# Autodesk Inventor assembly: panTiltSystemRB02
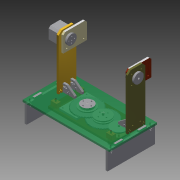
[picture p0: Inventor's stored thumbnail of the model, 180x180]
Saved by Autodesk Inventor 2013 (Build 170138000, 138)
## iProperties
Created: 2014-06-24
Part Number: panTiltSystemRB02
Document SubType Name: Assembly
Designer: Nano
Author: Nano
## Documents named in this file (23)
- C:\Users\Nano\Documents\InventorByron\InventorMasterProject\panTiltSystem\panTiltSystemRB02.iam
- C:\Users\Nano\Documents\InventorByron\InventorMasterProject\panTiltSystem\baseBoxShortSideRB01.ipt
- C:\Users\Nano\Documents\InventorByron\InventorMasterProject\panTiltSystem\panStepperMountRB01.ipt
- C:\Users\Nano\Documents\InventorByron\InventorMasterProject\panTiltSystem\stepper42BYGH007_RB01.ipt
- C:\Users\Nano\Documents\InventorByron\InventorMasterProject\panTiltSystem\tiltStructureCrossBeamRB01.ipt
- C:\Users\Nano\Documents\InventorByron\InventorMasterProject\panTiltSystem\tiltColumnStepperSide02_RB01.ipt
- C:\Users\Nano\Documents\InventorByron\InventorMasterProject\panTiltSystem\tiltColumnNonStepperSide02_RB01.ipt
- C:\Users\Nano\Documents\InventorByron\InventorMasterProject\panTiltSystem\projectorMountSide_RB01.ipt
- C:\Users\Nano\Documents\InventorByron\InventorMasterProject\panTiltSystem\projectorMountingBase_RB01.ipt
- C:\Users\Nano\Documents\InventorByron\InventorMasterProject\panTiltSystem\stepperShaftCollar_RB01.ipt
- C:\Users\Nano\Documents\InventorByron\InventorMasterProject\panTiltSystem\projectorMountOppositeSide_RB01.ipt
- C:\Users\Nano\Documents\InventorByron\InventorMasterProject\panTiltSystem\rotatingSupportShaft_RB01.ipt
- C:\Users\Nano\Documents\InventorByron\InventorMasterProject\panTiltSystem\shaftEndPlate_RB01.ipt
- C:\Users\Nano\Documents\InventorByron\InventorMasterProject\panTiltSystem\aaxaProjector01_RB01.ipt
- C:\Users\Nano\Documents\InventorByron\InventorMasterProject\panTiltSystem\cornerBraceV01.ipt
- C:\Users\Nano\Documents\InventorByron\InventorMasterProject\panTiltSystem\gearExperiments\gearTry01.iam
- C:\Users\Nano\Documents\InventorByron\InventorMasterProject\panTiltSystem\panGearShaft1.ipt
- C:\Users\Nano\Documents\InventorByron\InventorMasterProject\panTiltSystem\panGearSpacerBlocks.ipt
- C:\Users\Nano\Documents\InventorByron\InventorMasterProject\panTiltSystem\gearSpacerDisc01.ipt
- C:\Users\Nano\Documents\InventorByron\InventorMasterProject\panTiltSystem\gearGuideDiscOutputStage1.ipt
- C:\Users\Nano\Documents\InventorByron\InventorMasterProject\panTiltSystem\gearSpacerSmallOutputStage.ipt
- C:\Users\Nano\Documents\InventorByron\InventorMasterProject\panTiltSystem\panTilt_RB02_cutFiles\cutFiles125\driveGearCap.ipt
- C:\Users\Nano\Documents\InventorByron\InventorMasterProject\panTiltSystem\panTilt_RB02_cutFiles\cutFiles125\outputGearSupport.ipt
## Components (35 placed, 22 different names)
1. baseBoxShortSideRB01:1 — Mate:2, Flush:3, Mate:4
2. baseBoxShortSideRB01:2 — Mate:1, Mate:1, Flush:2
3. panStepperMountRB01:1 — Mate:1, Mate:1, Flush:2, Mate:2, Flush:3, Mate:4, Mate:7, Mate:60, Mate:61, Angle:6, Mate:64, Mate:72, Flush:27, Flush:28
4. stepper42BYGH007_RB01:1 — Mate:9, Mate:10, Mate:12, Mate:25, Mate:28, Mate:29, Mate:31, Mate:33
5. stepper42BYGH007_RB01:2 — zeroPositionPan, zeroPositionTilt, Mate:62, Mate:63
6. tiltStructureCrossBeamRB01:1 — Mate:7, Flush:5, Mate:8, Flush:6, Mate:11, Flush:7, Mate:15, Mate:18, Mate:21, Mate:24, Mate:48, Mate:50, Mate:51, Mate:54, Mate:56
7. tiltColumnStepperSide02_RB01:1 — Flush:5, Mate:8, Flush:6, Mate:9, Mate:10, Mate:28, Mate:32, Mate:49, Mate:52, Mate:53
8. tiltColumnNonStepperSide02_RB01:1 — Mate:11, Mate:12, Flush:7, Mate:39, zeroPositionPan, Mate:55, Mate:57, Mate:58, Mate:59
9. cornerBraceV01:1 — Mate:48, Mate:49, Flush:17
10. cornerBraceV01:2 — Mate:51, Mate:52, Flush:18
11. cornerBraceV01:3 — Mate:54, Mate:55, Flush:20
12. cornerBraceV01:4 — Mate:56, Mate:57, Flush:19
13. projectorMountSide_RB01:1 — Mate:31, Mate:32, Mate:34, Mate:35, Mate:36, Flush:14, Mate:37, Angle:1, Angle:2, Flush:15, Flush:16
14. projectorMountingBase_RB01:1 — Flush:13, Mate:36, Flush:14, Mate:37, Angle:1, Mate:38, Mate:46, Angle:3, Mate:47, zeroPositionTilt
15. stepperShaftCollar_RB01:1 — Mate:29, Mate:25, Mate:33, Mate:34, Mate:35
16. projectorMountOppositeSide_RB01:1 — Mate:38, Angle:2, Flush:15, Flush:16, Mate:44
17. rotatingSupportShaft_RB01:1 — Mate:39, Mate:40, Mate:41, Mate:42, Mate:43
18. shaftEndPlate_RB01:1 — Mate:40, Mate:42, Mate:44
19. shaftEndPlate_RB01:2 — Mate:41, Mate:43
20. aaxaProjector01_RB01:1 — Mate:46, Angle:3, Mate:47
21. gearTry01:1 [sub-assembly] — Mate:60, Mate:61, Angle:6, Mate:62, Mate:63, Flush:21, Flush:22, Flush:23, Flush:24, Mate:65, Mate:66, Angle:7, Mate:67, Mate:68, Angle:8, Mate:69, Mate:70, Angle:9, Flush:25, Flush:26, Mate:74, Mate:75, Mate:76, Mate:77, Flush:31, Flush:32, Flush:33, Flush:34
22. panGearShaft1:1 — Flush:21, Flush:22, Mate:71
23. panGearSpacerBlocks:1 — Flush:23, Flush:24, Mate:64
24. panGearSpacerBlocks:2 — Mate:65, Mate:66, Angle:7
25. panGearSpacerBlocks:3 — Mate:67, Mate:68, Angle:8
26. panGearSpacerBlocks:4 — Mate:69, Mate:70, Angle:9
27. gearSpacerDisc01:1 — Flush:25, Flush:26
28. gearSpacerDisc01:2 — Mate:71, Mate:72
29. gearGuideDiscOutputStage1:1 — Flush:27, Flush:28, Mate:73
30. gearSpacerDisc01:3 — Mate:73, Mate:74
31. gearSpacerDisc01:4 — Mate:75, Mate:76, Flush:29, Flush:30
32. gearSpacerSmallOutputStage:1 — Flush:29, Flush:30
33. panGearShaft1:2 — Mate:77, Flush:31
34. driveGearCap:1 — Flush:32
35. outputGearSupport:1 — Flush:33, Flush:34
## Relationships (102: Mate 63, Flush 30, Angle 9)
- Mate:1: baseBoxShortSideRB01:2 ↔ panStepperMountRB01:1
- Mate:1: baseBoxShortSideRB01:2 ↔ panStepperMountRB01:1
- Flush:2: baseBoxShortSideRB01:2 ↔ panStepperMountRB01:1
- Mate:2: baseBoxShortSideRB01:1 ↔ panStepperMountRB01:1
- Flush:3: baseBoxShortSideRB01:1 ↔ panStepperMountRB01:1
- Mate:4: baseBoxShortSideRB01:1 ↔ panStepperMountRB01:1
- Mate:7 (1.016 mm): panStepperMountRB01:1 ↔ tiltStructureCrossBeamRB01:1
- Flush:5: tiltStructureCrossBeamRB01:1 ↔ tiltColumnStepperSide02_RB01:1
- Mate:8: tiltStructureCrossBeamRB01:1 ↔ tiltColumnStepperSide02_RB01:1
- Flush:6: tiltStructureCrossBeamRB01:1 ↔ tiltColumnStepperSide02_RB01:1
- Mate:9: stepper42BYGH007_RB01:1 ↔ tiltColumnStepperSide02_RB01:1
- Mate:10: stepper42BYGH007_RB01:1 ↔ tiltColumnStepperSide02_RB01:1
- Mate:11: tiltStructureCrossBeamRB01:1 ↔ tiltColumnNonStepperSide02_RB01:1
- Mate:12: stepper42BYGH007_RB01:1 ↔ tiltColumnNonStepperSide02_RB01:1
- Flush:7: tiltStructureCrossBeamRB01:1 ↔ tiltColumnNonStepperSide02_RB01:1
- Mate:15: tiltStructureCrossBeamRB01:1
- [Flush] (-3.175 mm): cornerBraceV01:2
- Mate:18: tiltStructureCrossBeamRB01:1
- [Flush] (-3.175 mm): cornerBraceV01:3
- Mate:21: tiltStructureCrossBeamRB01:1
- [Flush] (-3.175 mm): cornerBraceV01:4
- Mate:24: tiltStructureCrossBeamRB01:1
- Mate:25: stepper42BYGH007_RB01:1 ↔ stepperShaftCollar_RB01:1
- Flush:13 (1.8542 mm): projectorMountingBase_RB01:1
- Mate:28: stepper42BYGH007_RB01:1 ↔ tiltColumnStepperSide02_RB01:1
- Mate:29: stepper42BYGH007_RB01:1 ↔ stepperShaftCollar_RB01:1
- Mate:31: stepper42BYGH007_RB01:1 ↔ projectorMountSide_RB01:1
- Mate:32 (1.016 mm): tiltColumnStepperSide02_RB01:1 ↔ projectorMountSide_RB01:1
- Mate:33: stepper42BYGH007_RB01:1 ↔ stepperShaftCollar_RB01:1
- Mate:34: projectorMountSide_RB01:1 ↔ stepperShaftCollar_RB01:1
- Mate:35: projectorMountSide_RB01:1 ↔ stepperShaftCollar_RB01:1
- Mate:36: projectorMountSide_RB01:1 ↔ projectorMountingBase_RB01:1
- Flush:14: projectorMountSide_RB01:1 ↔ projectorMountingBase_RB01:1
- Mate:37 (-3.175 mm): projectorMountSide_RB01:1 ↔ projectorMountingBase_RB01:1
- Angle:1 (0 deg): projectorMountSide_RB01:1 ↔ projectorMountingBase_RB01:1
- Mate:38: projectorMountingBase_RB01:1 ↔ projectorMountOppositeSide_RB01:1
- Angle:2 (0 deg): projectorMountSide_RB01:1 ↔ projectorMountOppositeSide_RB01:1
- Flush:15: projectorMountSide_RB01:1 ↔ projectorMountOppositeSide_RB01:1
- Flush:16: projectorMountSide_RB01:1 ↔ projectorMountOppositeSide_RB01:1
- Mate:39: tiltColumnNonStepperSide02_RB01:1 ↔ rotatingSupportShaft_RB01:1
- Mate:40: rotatingSupportShaft_RB01:1 ↔ shaftEndPlate_RB01:1
- Mate:41: rotatingSupportShaft_RB01:1 ↔ shaftEndPlate_RB01:2
- Mate:42: rotatingSupportShaft_RB01:1 ↔ shaftEndPlate_RB01:1
- Mate:43: rotatingSupportShaft_RB01:1 ↔ shaftEndPlate_RB01:2
- Mate:44 (1.016 mm): projectorMountOppositeSide_RB01:1 ↔ shaftEndPlate_RB01:1
- Mate:46: projectorMountingBase_RB01:1 ↔ aaxaProjector01_RB01:1
- Angle:3 (0 deg): projectorMountingBase_RB01:1 ↔ aaxaProjector01_RB01:1
- Mate:47: projectorMountingBase_RB01:1 ↔ aaxaProjector01_RB01:1
- Mate:48: tiltStructureCrossBeamRB01:1 ↔ cornerBraceV01:1
- Mate:49: tiltColumnStepperSide02_RB01:1 ↔ cornerBraceV01:1
- Flush:17 (-3.175 mm): cornerBraceV01:1
- zeroPositionPan [Angle] (0 deg): stepper42BYGH007_RB01:2 ↔ tiltColumnNonStepperSide02_RB01:1
- zeroPositionTilt [Angle] (0 deg): stepper42BYGH007_RB01:2 ↔ projectorMountingBase_RB01:1
- Mate:50: tiltStructureCrossBeamRB01:1
- Mate:51: tiltStructureCrossBeamRB01:1 ↔ cornerBraceV01:2
- Mate:52: tiltColumnStepperSide02_RB01:1 ↔ cornerBraceV01:2
- Flush:18 (-3.175 mm): cornerBraceV01:2
- Mate:53: tiltColumnStepperSide02_RB01:1
- Mate:54: tiltStructureCrossBeamRB01:1 ↔ cornerBraceV01:3
- Mate:55: tiltColumnNonStepperSide02_RB01:1 ↔ cornerBraceV01:3
- Mate:56: tiltStructureCrossBeamRB01:1 ↔ cornerBraceV01:4
- Mate:57: tiltColumnNonStepperSide02_RB01:1 ↔ cornerBraceV01:4
- Flush:19 (-3.175 mm): cornerBraceV01:4
- Flush:20 (-3.175 mm): cornerBraceV01:3
- Mate:58: tiltColumnNonStepperSide02_RB01:1
- Mate:59: tiltColumnNonStepperSide02_RB01:1
- Mate:60: panStepperMountRB01:1 ↔ gearTry01:1
- Mate:61 (3.175 mm): panStepperMountRB01:1 ↔ gearTry01:1
- Angle:6 (0 deg): panStepperMountRB01:1 ↔ gearTry01:1
- Mate:62: stepper42BYGH007_RB01:2 ↔ gearTry01:1
- Mate:63: stepper42BYGH007_RB01:2 ↔ gearTry01:1
- Flush:21: gearTry01:1 ↔ panGearShaft1:1
- Flush:22: gearTry01:1 ↔ panGearShaft1:1
- Flush:23: gearTry01:1 ↔ panGearSpacerBlocks:1
- Flush:24: gearTry01:1 ↔ panGearSpacerBlocks:1
- Mate:64: panStepperMountRB01:1 ↔ panGearSpacerBlocks:1
- Mate:65: gearTry01:1 ↔ panGearSpacerBlocks:2
- Mate:66: gearTry01:1 ↔ panGearSpacerBlocks:2
- Angle:7 (0 deg): gearTry01:1 ↔ panGearSpacerBlocks:2
- Mate:67: gearTry01:1 ↔ panGearSpacerBlocks:3
- Mate:68: gearTry01:1 ↔ panGearSpacerBlocks:3
- Angle:8 (0 deg): gearTry01:1 ↔ panGearSpacerBlocks:3
- Mate:69: gearTry01:1 ↔ panGearSpacerBlocks:4
- Mate:70: gearTry01:1 ↔ panGearSpacerBlocks:4
- Angle:9 (0 deg): gearTry01:1 ↔ panGearSpacerBlocks:4
- Flush:25: gearTry01:1 ↔ gearSpacerDisc01:1
- Flush:26: gearTry01:1 ↔ gearSpacerDisc01:1
- Mate:71: panGearShaft1:1 ↔ gearSpacerDisc01:2
- Mate:72: panStepperMountRB01:1 ↔ gearSpacerDisc01:2
- Flush:27: panStepperMountRB01:1 ↔ gearGuideDiscOutputStage1:1
- Flush:28: panStepperMountRB01:1 ↔ gearGuideDiscOutputStage1:1
- Mate:73: gearGuideDiscOutputStage1:1 ↔ gearSpacerDisc01:3
- Mate:74: gearTry01:1 ↔ gearSpacerDisc01:3
- Mate:75: gearTry01:1 ↔ gearSpacerDisc01:4
- Mate:76: gearTry01:1 ↔ gearSpacerDisc01:4
- Flush:29: gearSpacerDisc01:4 ↔ gearSpacerSmallOutputStage:1
- Flush:30: gearSpacerDisc01:4 ↔ gearSpacerSmallOutputStage:1
- Mate:77: gearTry01:1 ↔ panGearShaft1:2
- Flush:31: gearTry01:1 ↔ panGearShaft1:2
- Flush:32: gearTry01:1 ↔ driveGearCap:1
- Flush:33: gearTry01:1 ↔ outputGearSupport:1
- Flush:34: gearTry01:1 ↔ outputGearSupport:1
